# Autodesk Inventor assembly: snow_can_assembly
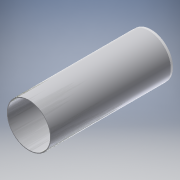
[picture p0: Inventor's stored thumbnail of the model, 180x180]
Saved by Autodesk Inventor 2016 (Build 200138000, 138)
## iProperties
Created: 2017-01-14
Part Number: snow_can_assembly
Document SubType Name: Assembly
Designer: hesaon
Author: hesaon
## Documents named in this file (3)
- D:\documents\SOD-II\cad\snow_can\snow_can_assembly.iam
- D:\documents\SOD-II\cad\snow_can\snow_can_bottom.ipt
- D:\documents\SOD-II\cad\snow_can\snow_can_middle.ipt
## Components (2 placed, 2 different names)
1. snow_can_bottom:1 — Insert:1
2. snow_can_middle:1 — Insert:1
## Relationships (1: Insert 1)
- Insert:1: snow_can_bottom:1 ↔ snow_can_middle:1
